# Autodesk Inventor assembly: [Midterm]Design
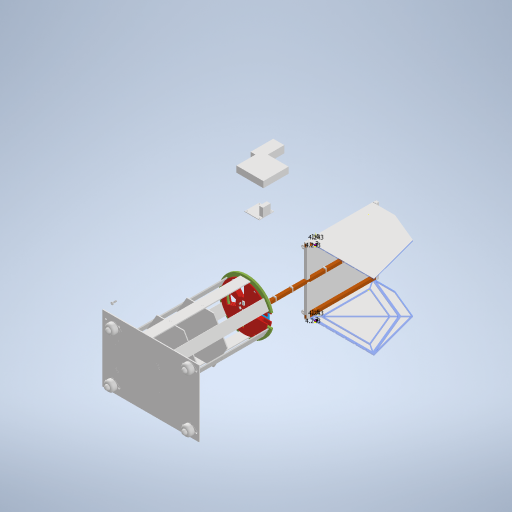
[picture p0: Inventor's stored thumbnail of the model, 512x512]
Saved by Autodesk Inventor 2024.2 (Build 282272000, 272)
## iProperties
Created: 2024-04-09
Part Number: [Midterm]Design
Document SubType Name: Assembly
Designer: USER
Author: USER
## Documents named in this file (23)
- C:\Users\user\Documents\機械工程實務\Practice-of-Mechanical-Engineering\3D_CAD_Drawing\[Midterm]Design\[Midterm]Design.iam
- C:\Users\user\Documents\機械工程實務\Practice-of-Mechanical-Engineering\3D_CAD_Drawing\[Midterm]Design\cow_wheel.ipt
- C:\Users\user\Documents\機械工程實務\Practice-of-Mechanical-Engineering\3D_CAD_Drawing\[Midterm]Design\back_down_hold.ipt
- C:\Users\user\Documents\機械工程實務\Practice-of-Mechanical-Engineering\3D_CAD_Drawing\[Midterm]Design\back_cir_hold.ipt
- C:\Users\user\Documents\機械工程實務\Practice-of-Mechanical-Engineering\3D_CAD_Drawing\[Midterm]Design\middle_space.ipt
- C:\Users\user\Documents\機械工程實務\Practice-of-Mechanical-Engineering\3D_CAD_Drawing\[Midterm]Design\rolling_plate.ipt
- C:\Users\user\Documents\機械工程實務\Practice-of-Mechanical-Engineering\3D_CAD_Drawing\[Midterm]Design\rolling_plate_top.ipt
- C:\Users\user\Documents\機械工程實務\Practice-of-Mechanical-Engineering\3D_CAD_Drawing\[Midterm]Design\rolling_plate_small.ipt
- C:\Users\user\Documents\機械工程實務\Practice-of-Mechanical-Engineering\3D_CAD_Drawing\[Midterm]Design\左右.ipt
- C:\Users\user\Documents\機械工程實務\Practice-of-Mechanical-Engineering\3D_CAD_Drawing\[Midterm]Design\左右2.ipt
- C:\Users\user\Documents\機械工程實務\Practice-of-Mechanical-Engineering\3D_CAD_Drawing\[Midterm]Design\馬達.ipt
- C:\Users\user\Documents\機械工程實務\Practice-of-Mechanical-Engineering\3D_CAD_Drawing\[Midterm]Design\軸.ipt
- C:\Users\user\Documents\機械工程實務\Practice-of-Mechanical-Engineering\3D_CAD_Drawing\[Midterm]Design\螺絲.ipt
- C:\Users\user\Documents\機械工程實務\Practice-of-Mechanical-Engineering\3D_CAD_Drawing\[Midterm]Design\Base_final.ipt
- C:\Users\user\Documents\機械工程實務\Practice-of-Mechanical-Engineering\3D_CAD_Drawing\[Midterm]Design\sail(Midterm).iam
- C:\Users\user\Documents\機械工程實務\Practice-of-Mechanical-Engineering\3D_CAD_Drawing\[Midterm]Design\插銷B.ipt
- C:\Users\user\Documents\機械工程實務\Practice-of-Mechanical-Engineering\3D_CAD_Drawing\[Midterm]Design\插銷A.ipt
- C:\Users\user\Documents\機械工程實務\Practice-of-Mechanical-Engineering\3D_CAD_Drawing\[Midterm]Design\9V方型電池盒.ipt
- C:\Users\user\Documents\機械工程實務\Practice-of-Mechanical-Engineering\3D_CAD_Drawing\[Midterm]Design\18650電池盒.ipt
- C:\Users\user\Documents\機械工程實務\Practice-of-Mechanical-Engineering\3D_CAD_Drawing\[Midterm]Design\Arduino板.ipt
- C:\Users\user\Documents\機械工程實務\Practice-of-Mechanical-Engineering\3D_CAD_Drawing\[Midterm]Design\馬達驅動模組.ipt
- C:\Users\user\Documents\機械工程實務\Practice-of-Mechanical-Engineering\3D_CAD_Drawing\[Midterm]Design\麵包板.ipt
- C:\Users\user\Documents\機械工程實務\Practice-of-Mechanical-Engineering\3D_CAD_Drawing\[Midterm]Design\m4螺栓\m4螺栓.ipt
## Components (44 placed, 22 different names)
1. cow_wheel:1 — 貼合:82, 貼合:83, 貼合:84
2. cow_wheel:2 — 貼合:86
3. cow_wheel:3 — 貼合:80, 貼合:81, 貼合:85
4. cow_wheel:4 — 貼合:75, 貼合:76, 貼合:77, 貼合:78, 貼合:79
5. back_down_hold:1 — 貼合:99, 貼合:100, 貼合:101, 貼合:102
6. back_down_hold:2 — 貼合:34, 齊平:14, 相切:1, 齊平:28, 貼合:92, 貼合:93, 貼合:94
7. back_down_hold:3 — 齊平:5, 貼合:47, 齊平:13, 貼合:90, 貼合:91
8. back_down_hold:4 — 貼合:87, 貼合:97, 貼合:98
9. back_down_hold:5 — 齊平:6, 貼合:46, 齊平:12, 貼合:48, 貼合:88, 貼合:89, 貼合:105
10. back_down_hold:6 — 齊平:5, 齊平:6, 貼合:32, 貼合:33, 貼合:95, 貼合:96
11. back_cir_hold:1 — 貼合:32, 貼合:33, 貼合:34, 貼合:104, 角度:1, 貼合:109
12. middle_space:1 — 齊平:13, 貼合:48, 齊平:14, 齊平:28
13. middle_space:2 — 貼合:46, 齊平:12, 貼合:47
14. rolling_plate:2 — 貼合:56, 貼合:57, 齊平:24, 貼合:104, 貼合:108, 貼合:109, 齊平:31, 貼合:135, 貼合:136, 貼合:139, 貼合:140, 貼合:141
15. rolling_plate_top:1 — 相切:1, 貼合:58, 貼合:59, 貼合:60, 貼合:61, 貼合:62, 貼合:63, 角度:1, 貼合:108, 貼合:113, 貼合:114, 貼合:115, 貼合:116, 貼合:117, 齊平:30, 貼合:118, 貼合:119, 貼合:120, 貼合:121, 貼合:122, 貼合:123, 貼合:124, 貼合:125, 貼合:126, 貼合:128, 貼合:129, 貼合:131, 貼合:132, 貼合:133, 貼合:137
16. rolling_plate_small:1 — 貼合:52, 齊平:16, 齊平:19, 貼合:56, 齊平:24
17. rolling_plate_small:2 — 貼合:52, 齊平:16, 齊平:19, 貼合:57, 貼合:107, 齊平:29
18. rolling_plate_small:4 — 貼合:107, 齊平:29, 貼合:116, 貼合:117, 齊平:30
19. 左右:1 — 貼合:58, 貼合:59, 貼合:60, 貼合:66, 貼合:67, 齊平:26, 貼合:68, 齊平:27
20. 左右2:1 — 貼合:61, 貼合:62, 貼合:63, 角度:2
21. 馬達:1 — 貼合:64, 貼合:65, 貼合:69, 貼合:70, 貼合:71
22. 軸:1 — 貼合:64, 貼合:65, 貼合:110, 貼合:111, 貼合:112
23. 螺絲:1 — 齊平:25, 貼合:66, 貼合:67, 齊平:26, 貼合:69, 貼合:70
24. 螺絲:2 — 齊平:25, 貼合:68, 齊平:27, 貼合:71
25. Base_final:1 — 貼合:75, 貼合:76, 貼合:77, 貼合:78, 貼合:79, 貼合:80, 貼合:81, 貼合:82, 貼合:83, 貼合:84, 貼合:85, 貼合:86, 貼合:87, 貼合:88, 貼合:89, 貼合:90, 貼合:91, 貼合:92, 貼合:93, 貼合:94, 貼合:95, 貼合:96, 貼合:97, 貼合:98, 貼合:99, 貼合:100, 貼合:101, 貼合:102, 貼合:105, 齊平:40, 貼合:142, 貼合:143, 齊平:41, 齊平:42
26. sail(Midterm):1 [sub-assembly] — 貼合:110, 貼合:111, 貼合:112, 角度:2
27. 插銷A:1 — 齊平:32, 貼合:127, 齊平:33, 貼合:128
28. 插銷B:2 — 貼合:123, 貼合:124, 貼合:125
29. 插銷A:2 — 貼合:138, 齊平:38, 齊平:39, 貼合:141
30. 插銷B:3 — 貼合:121, 齊平:31, 貼合:122
31. 插銷A:3 — 貼合:130, 齊平:34, 齊平:35, 貼合:131
32. 插銷B:4 — 貼合:118, 貼合:119, 貼合:120
33. 插銷A:5 — 貼合:126, 齊平:32, 貼合:127, 齊平:33, 貼合:129
34. 插銷B:6 — 貼合:113, 貼合:114, 貼合:115
35. 插銷A:6 — 貼合:134, 齊平:36, 齊平:37, 貼合:135, 貼合:136
36. 插銷A:7 — 貼合:130, 齊平:34, 齊平:35, 貼合:132, 貼合:133
37. 插銷A:8 — 貼合:138, 齊平:38, 齊平:39, 貼合:139, 貼合:140
38. 插銷A:9 — 貼合:134, 齊平:36, 齊平:37, 貼合:137
39. 9V方型電池盒:1
40. 18650電池盒:1
41. Arduino板:1 — 貼合:143, 齊平:41, 齊平:42, 齊平:43
42. 馬達驅動模組:1
43. 麵包板:1 — 齊平:40, 貼合:142, 齊平:43
44. m4螺栓:1
## Relationships (120: Mate 90, Flush 27, Angle 2, Tangent 1)
- 齊平:5 [Flush]: back_down_hold:3 ↔ back_down_hold:6
- 齊平:6 [Flush]: back_down_hold:5 ↔ back_down_hold:6
- 貼合:32 [Mate]: back_down_hold:6 ↔ back_cir_hold:1
- 貼合:33 [Mate]: back_down_hold:6 ↔ back_cir_hold:1
- 貼合:34 [Mate]: back_down_hold:2 ↔ back_cir_hold:1
- 貼合:46 [Mate]: back_down_hold:5 ↔ middle_space:2
- 齊平:12 [Flush]: back_down_hold:5 ↔ middle_space:2
- 貼合:47 [Mate]: back_down_hold:3 ↔ middle_space:2
- 齊平:13 [Flush]: back_down_hold:3 ↔ middle_space:1
- 貼合:48 [Mate]: back_down_hold:5 ↔ middle_space:1
- 齊平:14 [Flush]: back_down_hold:2 ↔ middle_space:1
- 相切:1 [Tangent]: back_down_hold:2 ↔ rolling_plate_top:1
- 貼合:52 [Mate]: rolling_plate_small:1 ↔ rolling_plate_small:2
- 齊平:16 [Flush]: rolling_plate_small:1 ↔ rolling_plate_small:2
- 齊平:19 [Flush]: rolling_plate_small:1 ↔ rolling_plate_small:2
- 貼合:56 [Mate]: rolling_plate:2 ↔ rolling_plate_small:1
- 貼合:57 [Mate]: rolling_plate:2 ↔ rolling_plate_small:2
- 齊平:24 [Flush]: rolling_plate:2 ↔ rolling_plate_small:1
- 貼合:58 [Mate]: rolling_plate_top:1 ↔ 左右:1
- 貼合:59 [Mate]: rolling_plate_top:1 ↔ 左右:1
- 貼合:60 [Mate]: rolling_plate_top:1 ↔ 左右:1
- 貼合:61 [Mate]: rolling_plate_top:1 ↔ 左右2:1
- 貼合:62 [Mate]: rolling_plate_top:1 ↔ 左右2:1
- 貼合:63 [Mate]: rolling_plate_top:1 ↔ 左右2:1
- 貼合:64 [Mate]: 馬達:1 ↔ 軸:1
- 貼合:65 [Mate]: 馬達:1 ↔ 軸:1
- 齊平:25 [Flush]: 螺絲:1 ↔ 螺絲:2
- 貼合:66 [Mate]: 左右:1 ↔ 螺絲:1
- 貼合:67 [Mate]: 左右:1 ↔ 螺絲:1
- 齊平:26 [Flush]: 左右:1 ↔ 螺絲:1
- 貼合:68 [Mate]: 左右:1 ↔ 螺絲:2
- 齊平:27 [Flush]: 左右:1 ↔ 螺絲:2
- 貼合:69 [Mate]: 馬達:1 ↔ 螺絲:1
- 貼合:70 [Mate]: 馬達:1 ↔ 螺絲:1
- 貼合:71 [Mate]: 馬達:1 ↔ 螺絲:2
- 齊平:28 [Flush]: back_down_hold:2 ↔ middle_space:1
- 貼合:75 [Mate]: cow_wheel:4 ↔ Base_final:1
- 貼合:76 [Mate]: cow_wheel:4 ↔ Base_final:1
- 貼合:77 [Mate]: cow_wheel:4 ↔ Base_final:1
- 貼合:78 [Mate]: cow_wheel:4 ↔ Base_final:1
- 貼合:79 [Mate]: cow_wheel:4 ↔ Base_final:1
- 貼合:80 [Mate]: cow_wheel:3 ↔ Base_final:1
- 貼合:81 [Mate]: cow_wheel:3 ↔ Base_final:1
- 貼合:82 [Mate]: cow_wheel:1 ↔ Base_final:1
- 貼合:83 [Mate]: cow_wheel:1 ↔ Base_final:1
- 貼合:84 [Mate]: cow_wheel:1 ↔ Base_final:1
- 貼合:85 [Mate]: cow_wheel:3 ↔ Base_final:1
- 貼合:86 [Mate]: cow_wheel:2 ↔ Base_final:1
- 貼合:87 [Mate]: back_down_hold:4 ↔ Base_final:1
- 貼合:88 [Mate]: back_down_hold:5 ↔ Base_final:1
- 貼合:89 [Mate]: back_down_hold:5 ↔ Base_final:1
- 貼合:90 [Mate]: back_down_hold:3 ↔ Base_final:1
- 貼合:91 [Mate]: back_down_hold:3 ↔ Base_final:1
- 貼合:92 [Mate]: back_down_hold:2 ↔ Base_final:1
- 貼合:93 [Mate]: back_down_hold:2 ↔ Base_final:1
- 貼合:94 [Mate]: back_down_hold:2 ↔ Base_final:1
- 貼合:95 [Mate]: back_down_hold:6 ↔ Base_final:1
- 貼合:96 [Mate]: back_down_hold:6 ↔ Base_final:1
- 貼合:97 [Mate]: back_down_hold:4 ↔ Base_final:1
- 貼合:98 [Mate]: back_down_hold:4 ↔ Base_final:1
- 貼合:99 [Mate]: back_down_hold:1 ↔ Base_final:1
- 貼合:100 [Mate]: back_down_hold:1 ↔ Base_final:1
- 貼合:101 [Mate]: back_down_hold:1 ↔ Base_final:1
- 貼合:102 [Mate]: back_down_hold:1 ↔ Base_final:1
- 貼合:104 [Mate]: back_cir_hold:1 ↔ rolling_plate:2
- 貼合:105 [Mate]: back_down_hold:5 ↔ Base_final:1
- 角度:1 [Angle] (0 deg): back_cir_hold:1 ↔ rolling_plate_top:1
- 貼合:107 [Mate]: rolling_plate_small:2 ↔ rolling_plate_small:4
- 貼合:108 [Mate]: rolling_plate:2 ↔ rolling_plate_top:1
- 齊平:29 [Flush]: rolling_plate_small:2 ↔ rolling_plate_small:4
- 貼合:109 [Mate] (1.5 mm): back_cir_hold:1 ↔ rolling_plate:2
- 貼合:110 [Mate]: 軸:1 ↔ sail(Midterm):1
- 貼合:111 [Mate]: 軸:1 ↔ sail(Midterm):1
- 貼合:112 [Mate]: 軸:1 ↔ sail(Midterm):1
- 貼合:113 [Mate]: rolling_plate_top:1 ↔ 插銷B:6
- 貼合:114 [Mate]: rolling_plate_top:1 ↔ 插銷B:6
- 貼合:115 [Mate]: rolling_plate_top:1 ↔ 插銷B:6
- 貼合:116 [Mate]: rolling_plate_top:1 ↔ rolling_plate_small:4
- 貼合:117 [Mate]: rolling_plate_top:1 ↔ rolling_plate_small:4
- 齊平:30 [Flush]: rolling_plate_top:1 ↔ rolling_plate_small:4
- 貼合:118 [Mate]: rolling_plate_top:1 ↔ 插銷B:4
- 貼合:119 [Mate]: rolling_plate_top:1 ↔ 插銷B:4
- 貼合:120 [Mate]: rolling_plate_top:1 ↔ 插銷B:4
- 貼合:121 [Mate]: rolling_plate_top:1 ↔ 插銷B:3
- 齊平:31 [Flush]: rolling_plate:2 ↔ 插銷B:3
- 貼合:122 [Mate]: rolling_plate_top:1 ↔ 插銷B:3
- 貼合:123 [Mate]: rolling_plate_top:1 ↔ 插銷B:2
- 貼合:124 [Mate]: rolling_plate_top:1 ↔ 插銷B:2
- 貼合:125 [Mate]: rolling_plate_top:1 ↔ 插銷B:2
- 貼合:126 [Mate]: rolling_plate_top:1 ↔ 插銷A:5
- 齊平:32 [Flush]: 插銷A:1 ↔ 插銷A:5
- 貼合:127 [Mate]: 插銷A:1 ↔ 插銷A:5
- 齊平:33 [Flush]: 插銷A:1 ↔ 插銷A:5
- 貼合:128 [Mate]: rolling_plate_top:1 ↔ 插銷A:1
- 貼合:129 [Mate]: rolling_plate_top:1 ↔ 插銷A:5
- 貼合:130 [Mate]: 插銷A:3 ↔ 插銷A:7
- 齊平:34 [Flush]: 插銷A:3 ↔ 插銷A:7
- 齊平:35 [Flush]: 插銷A:3 ↔ 插銷A:7
- 貼合:131 [Mate]: rolling_plate_top:1 ↔ 插銷A:3
- 貼合:132 [Mate]: rolling_plate_top:1 ↔ 插銷A:7
- 貼合:133 [Mate]: rolling_plate_top:1 ↔ 插銷A:7
- 貼合:134 [Mate]: 插銷A:6 ↔ 插銷A:9
- 齊平:36 [Flush]: 插銷A:6 ↔ 插銷A:9
- 齊平:37 [Flush]: 插銷A:6 ↔ 插銷A:9
- 貼合:135 [Mate]: rolling_plate:2 ↔ 插銷A:6
- 貼合:136 [Mate]: rolling_plate:2 ↔ 插銷A:6
- 貼合:137 [Mate]: rolling_plate_top:1 ↔ 插銷A:9
- 貼合:138 [Mate]: 插銷A:2 ↔ 插銷A:8
- 齊平:38 [Flush]: 插銷A:2 ↔ 插銷A:8
- 齊平:39 [Flush]: 插銷A:2 ↔ 插銷A:8
- 貼合:139 [Mate]: rolling_plate:2 ↔ 插銷A:8
- 貼合:140 [Mate]: rolling_plate:2 ↔ 插銷A:8
- 貼合:141 [Mate]: rolling_plate:2 ↔ 插銷A:2
- 角度:2 [Angle] (0 deg): 左右2:1 ↔ sail(Midterm):1
- 齊平:40 [Flush] (10 mm): Base_final:1 ↔ 麵包板:1
- 貼合:142 [Mate]: Base_final:1 ↔ 麵包板:1
- 貼合:143 [Mate]: Base_final:1 ↔ Arduino板:1
- 齊平:41 [Flush] (30 mm): Base_final:1 ↔ Arduino板:1
- 齊平:42 [Flush] (25 mm): Base_final:1 ↔ Arduino板:1
- 齊平:43 [Flush] (-5 mm): Arduino板:1 ↔ 麵包板:1
